# Autodesk Inventor assembly: SCS5-10
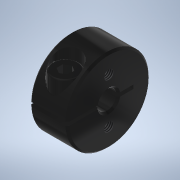
[picture p0: Inventor's stored thumbnail of the model, 180x180]
Saved by Autodesk Inventor 2022.3 (Build 263350000, 350)
## iProperties
Category: PARTsolutions
Company: MISUMI
Created: 2019-11-13
Part Number: SCS5-10
Catalog Web Link: www.cadenas.de
Description: SCS, PSCS, SSCS, SCSA, SCSAW, SCSAB-Set Collars - Slit - Standard Type
Vendor: MISUMI
Document SubType Name: Assembly
Designer: psadmin
Manufacturer: MISUMI
PSOL_IDENT_0: {$CADENAS_DATA\23d-libs\misumi\metric\03_set_collars\scs_asmtab.prj},200 {VTYP=3D},{STYP=ASSTAB},{NB=
PSOL_IDENT_1: SCS5-10},{LINA=SCS5-10},{NN=SCS, PSCS, SSCS, SCSA, SCSAW, SCSAB},{DATE=05.11.2019 07:45:28},{GEOMDAT
PSOL_IDENT_2: E=02.02.2011},{VERSION=},{LINEID=230},{WBVAR=MAT,ST,BS},{WBNUMERIC=BS}  {NB=SCS5-10},{LINA=SCS5-10},
PSOL_IDENT_3: {KT=DUMMY},{PN=SCS5-10},{TYPE=SCS},{MAT=1045},{ST=Black Oxide},{AC=Hexagon Socket Head Cap Screw 1 P
PSOL_IDENT_4: c.},{D=5},{BS=10},{BALG=8,10},{B0=8,10},{B1=8,10},{B2=8},{D1=22},{M=M4},{THMD=4},{THDMIN=3.242},{ST0='
PSOL_IDENT_5: Black Oxide','Black Oxide','Electroless Nickel Plating','Electroless Nickel Plating'},{DD=4.5},{R=3.
PSOL_IDENT_6: 75},{W=1.0},{X=6.5},{Y=4.0},{Z=6~7},{Z1=6.50},{P1=0},{C=0.5},{L=10},{PPATH=scs_templ.prj},{MATA=  '1
PSOL_IDENT_7: 045','S45C(1045 Steel)(1.1191_C45E (Ck45))','304','SUS304(304 Stainless Steel)(1.4301_X5CrNi18-10)','
PSOL_IDENT_8: 2017','A2017(2017 Aluminum)(EN AW-2017_AlCu4MgSi)'  }
NN: SCS, PSCS, SSCS, SCSA, SCSAW, SCSAB
NT: Set Collars - Slit - Standard Type
NB: SCS5-10
NBSYN: $PN.
LINA: SCS5-10
PN: SCS5-10
MAT: 1045 Carbon Steel
ST: Black Oxide
AC: Hexagon Socket Head Cap Screw 1 Pc.
D: 5
BS: 10
D1: 22
M: M4
DD: 4.5
R: 3.75
W: 1
X: 6.5
Y: 4
Z: 6~7
SUPPLIER: MISUMI
ARTICLENO: SCS5-10
BOMINFO: SCS5-10
CREATOR: CADENAS GmbH
Title: SCS5-10
Author: Cadenas PARTsolutions
Comments: Set Collars - Slit - Standard Type
## Documents named in this file (3)
- C:\Users\YusukeKunita\Documents\GrabCAD\Development\BasicParts\SetCollar\SCS5-10\SCS5-10.iam
- C:\Users\YusukeKunita\Documents\GrabCAD\Development\BasicParts\SetCollar\SCS5-10\SCS5-10b.ipt
- C:\Users\YusukeKunita\Documents\GrabCAD\Development\BasicParts\SetCollar\SCS5-10\Slotted head cap screw ISO 4762 - M4x10.ipt
## Components (2 placed, 2 different names)
1. SCS5-10b:1 — body_screw_Z@1 <-> IP1_Z@2, body_screw_YZ@1 <-> IP1_YZ@2
2. Slotted head cap screw ISO 4762 - M4x10:1 — body_screw_Z@1 <-> IP1_Z@2, body_screw_YZ@1 <-> IP1_YZ@2
## Relationships (2: Mate 1, Angle 1)
- body_screw_Z@1 <-> IP1_Z@2 [Mate]: SCS5-10b:1 ↔ Slotted head cap screw ISO 4762 - M4x10:1
- body_screw_YZ@1 <-> IP1_YZ@2 [Angle] (0 deg): SCS5-10b:1 ↔ Slotted head cap screw ISO 4762 - M4x10:1
